# Autodesk Inventor assembly: Air filter
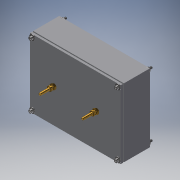
[picture p0: Inventor's stored thumbnail of the model, 180x180]
Saved by Autodesk Inventor 2018 (Build 220112000, 112)
## iProperties
Created: 2020-03-29
Part Number: Air filter
Document SubType Name: Assembly
Designer: emile
Author: emile
Title: LARGE PARTICUL FILTER
## Documents named in this file (6)
- C:\Users\emile\OneDrive\Documents\Inventor\Respirator\MultiLine\Air filter.iam
- C:\Users\emile\OneDrive\Documents\Inventor\Respirator\Peep\AirPressure\CorollaAirFilterCase.ipt
- C:\Users\emile\OneDrive\Documents\Inventor\Respirator\Peep\AirPressure\CorollaAirFilter.ipt
- C:\Users\emile\OneDrive\Documents\Inventor\Respirator\Peep\AirPressure\CorollaAirFilterCaseCover.ipt
- C:\Users\emile\OneDrive\Documents\Inventor\Respirator\Peep\AirPressure\Brass Barbed Hose Fitting for Air and Water.ipt
- C:\Users\emile\OneDrive\Documents\Inventor\Respirator\MultiLine\Air filter\Design Accelerator\Bolted Connection1.iam
## Components (10 placed, 5 different names)
1. CorollaAirFilterCase:1
2. CorollaAirFilter:1 — Mate:19
3. CorollaAirFilterCaseCover:1 — Mate:11, Mate:12, Mate:13, Mate:14, Mate:15, Mate:16, Mate:17, Mate:18, Mate:19
4. Brass Barbed Hose Fitting for Air and Water:1
5. Brass Barbed Hose Fitting for Air and Water:2
6. Brass Barbed Hose Fitting for Air and Water:3
7. Bolted Connection:1 [sub-assembly] — Mate:11, Mate:12
8. Bolted Connection:2 [sub-assembly] — Mate:15, Mate:18
9. Bolted Connection:3 [sub-assembly] — Mate:14, Mate:16
10. Bolted Connection:4 [sub-assembly] — Mate:13, Mate:17
## Relationships (20: Mate 18, Flush 2)
- [Mate]: CorollaAirFilterCase:1 ↔ CorollaAirFilter:1
- [Flush]: CorollaAirFilterCase:1 ↔ CorollaAirFilter:1
- [Mate]: CorollaAirFilterCase:1 ↔ CorollaAirFilter:1
- [Mate]: CorollaAirFilterCase:1 ↔ CorollaAirFilterCaseCover:1
- [Flush]: CorollaAirFilter:1 ↔ CorollaAirFilterCaseCover:1
- [Mate]: CorollaAirFilterCaseCover:1 ↔ Brass Barbed Hose Fitting for Air and Water:1
- [Mate]: CorollaAirFilterCaseCover:1 ↔ Brass Barbed Hose Fitting for Air and Water:1
- [Mate]: CorollaAirFilterCaseCover:1 ↔ Brass Barbed Hose Fitting for Air and Water:2
- [Mate]: CorollaAirFilterCaseCover:1 ↔ Brass Barbed Hose Fitting for Air and Water:2
- [Mate]: CorollaAirFilterCase:1 ↔ Brass Barbed Hose Fitting for Air and Water:3
- [Mate]: CorollaAirFilterCase:1 ↔ Brass Barbed Hose Fitting for Air and Water:3
- Mate:11: CorollaAirFilterCaseCover:1 ↔ Bolted Connection:1
- Mate:12: CorollaAirFilterCaseCover:1 ↔ Bolted Connection:1
- Mate:13: CorollaAirFilterCaseCover:1 ↔ Bolted Connection:4
- Mate:14: CorollaAirFilterCaseCover:1 ↔ Bolted Connection:3
- Mate:15: CorollaAirFilterCaseCover:1 ↔ Bolted Connection:2
- Mate:16: CorollaAirFilterCaseCover:1 ↔ Bolted Connection:3
- Mate:17: CorollaAirFilterCaseCover:1 ↔ Bolted Connection:4
- Mate:18: CorollaAirFilterCaseCover:1 ↔ Bolted Connection:2
- Mate:19: CorollaAirFilter:1 ↔ CorollaAirFilterCaseCover:1
